# Autodesk Inventor assembly: GalvoandK1s4
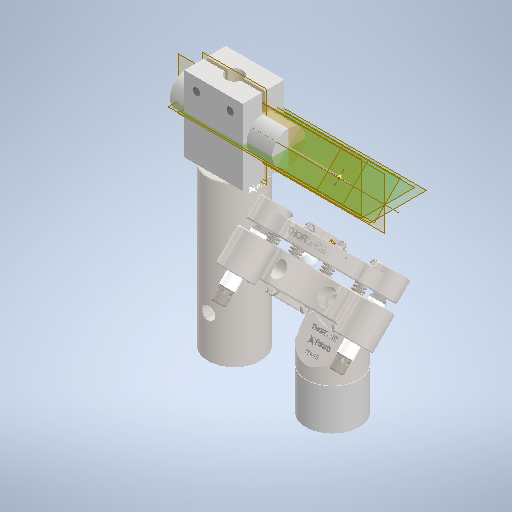
[picture p0: Inventor's stored thumbnail of the model, 512x512]
Saved by Autodesk Inventor 2025.2 (Build 292293000, 293)
## iProperties
Created: 2026-03-02
Part Number: GalvoandK1s4
Document SubType Name: Assembly
Designer: monolithic
Author: monolithic
## Documents named in this file (6)
- C:\Users\monolithic\Documents\GitHub\CAD\Monolith\John\Altair_PowellAndCylindricalBaseplatesCombined_10_16_2025\Assemblies\Subassemblies\GalvoandK1s4.iam
- C:\Users\monolithic\Documents\GitHub\navigate-hardware\downloads\ASLM_CTASLM_Baseplate\CAD Assemblies\Cylindrical ASLM\Galvo-Holder-PolarisMount_metal_v2.ipt
- C:\Users\monolithic\Documents\GitHub\navigate-hardware\downloads\ASLM_CTASLM_Baseplate\CAD Assemblies\Cylindrical ASLM\K1S4andMirrorNoPost.iam
- C:\Users\monolithic\Documents\GitHub\navigate-hardware\downloads\ASLM_CTASLM_Baseplate\CAD Assemblies\Cylindrical ASLM\Galvo_Galvo_Tilted.iam
- C:\Users\monolithic\Documents\GitHub\navigate-hardware\downloads\ASLM_CTASLM_Baseplate\CAD Assemblies\Cylindrical ASLM\PolarisPost_HeightAdjustment_0p77in_ForK1S4Mirrors_Machined.ipt
- C:\Users\monolithic\Documents\GitHub\navigate-hardware\downloads\ASLM_CTASLM_Baseplate\CAD Assemblies\Cylindrical ASLM\PLS-P3.ipt
## Components (5 placed, 5 different names)
1. Galvo-Holder-PolarisMount_metal_v2:1
2. K1S4andMirrorNoPost:1 [sub-assembly]
3. Galvo_Galvo_Tilted:1 [sub-assembly]
4. PolarisPost_HeightAdjustment_0p77in_ForK1S4Mirrors_Machined:1
5. PLS-P3:1
## Relationships (6: Mate 5, Angle 1)
- [Mate]: Galvo-Holder-PolarisMount_metal_v2:1 ↔ Galvo_Galvo_Tilted:1
- [Angle] (135 deg): Galvo-Holder-PolarisMount_metal_v2:1 ↔ Galvo_Galvo_Tilted:1
- [Mate]: K1S4andMirrorNoPost:1 ↔ PolarisPost_HeightAdjustment_0p77in_ForK1S4Mirrors_Machined:1
- [Mate]: K1S4andMirrorNoPost:1 ↔ PolarisPost_HeightAdjustment_0p77in_ForK1S4Mirrors_Machined:1
- [Mate]: Galvo-Holder-PolarisMount_metal_v2:1 ↔ PLS-P3:1
- [Mate]: Galvo-Holder-PolarisMount_metal_v2:1 ↔ PLS-P3:1
